# Autodesk Inventor assembly: Accelerator
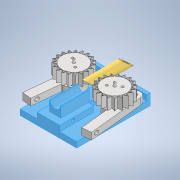
[picture p0: Inventor's stored thumbnail of the model, 180x180]
Saved by Autodesk Inventor 2021 (Build 250183000, 183)
## iProperties
Created: 2024-05-11
Part Number: Accelerator
Document SubType Name: Assembly
Designer: Lukas
Author: Lukas
## Documents named in this file (7)
- \\192.168.1.200\Storragepool\Datastorrage\CAD\Inventor 2019\Maccaroni-Gun\Inventor files\Accelerator.iam
- \\192.168.1.200\Storragepool\Datastorrage\CAD\Inventor 2019\Maccaroni-Gun\Inventor files\Motor_holder.ipt
- \\192.168.1.200\Storragepool\Datastorrage\CAD\Inventor 2019\Maccaroni-Gun\Inventor files\Motor_18mm.ipt
- \\192.168.1.200\Storragepool\Datastorrage\CAD\Inventor 2019\Maccaroni-Gun\Inventor files\Flywheel_base.ipt
- \\192.168.1.200\Storragepool\Datastorrage\CAD\Inventor 2019\Maccaroni-Gun\Inventor files\Antriebsrad.ipt
- \\192.168.1.200\Storragepool\Datastorrage\CAD\Inventor 2019\Maccaroni-Gun\Inventor files\Motor_holder_mirrored.ipt
- \\192.168.1.200\Storragepool\Datastorrage\CAD\Inventor 2019\Maccaroni-Gun\Inventor files\Maccaroni.ipt
## Components (8 placed, 6 different names)
1. Flywheel_base:1 — Mate:4, Mate:5, Mate:9, Mate:10, Mate:19, Angle:4, Angle:5, Flush:1, Flush:2, Flush:3
2. Motor_holder:1 — Mate:1, Mate:2, Mate:3, Mate:4, Mate:5, Rotation:1, Angle:4
3. Motor_holder_mirrored:1 — Mate:9, Mate:10, Mate:13, Mate:17, Mate:18, Rotation:1, Angle:5
4. Motor_18mm:1 — Mate:1, Mate:2, Mate:3, Mate:6, Mate:7, Mate:8
5. Motor_18mm:2 — Mate:13, Mate:14, Mate:15, Mate:16, Mate:17, Mate:18
6. Antriebsrad:1 — Mate:6, Mate:7, Mate:8
7. Antriebsrad:2 — Mate:14, Mate:15, Mate:16
8. Maccaroni:1 — Angle:3, Mate:19, Flush:4
## Relationships (25: Mate 17, Flush 4, Angle 3, RelateRotation 1)
- Mate:1: Motor_holder:1 ↔ Motor_18mm:1
- Mate:2: Motor_holder:1 ↔ Motor_18mm:1
- Mate:3: Motor_holder:1 ↔ Motor_18mm:1
- Mate:4: Flywheel_base:1 ↔ Motor_holder:1
- Mate:5: Flywheel_base:1 ↔ Motor_holder:1
- Mate:6: Motor_18mm:1 ↔ Antriebsrad:1
- Mate:7: Motor_18mm:1 ↔ Antriebsrad:1
- Mate:8: Motor_18mm:1 ↔ Antriebsrad:1
- Mate:9: Flywheel_base:1 ↔ Motor_holder_mirrored:1
- Mate:10: Flywheel_base:1 ↔ Motor_holder_mirrored:1
- Mate:13: Motor_holder_mirrored:1 ↔ Motor_18mm:2
- Mate:14: Motor_18mm:2 ↔ Antriebsrad:2
- Mate:15: Motor_18mm:2 ↔ Antriebsrad:2
- Mate:16: Motor_18mm:2 ↔ Antriebsrad:2
- Mate:17: Motor_holder_mirrored:1 ↔ Motor_18mm:2
- Mate:18: Motor_holder_mirrored:1 ↔ Motor_18mm:2
- Angle:3 (0 deg): Maccaroni:1
- Mate:19: Flywheel_base:1 ↔ Maccaroni:1
- Rotation:1 [RelateRotation] (1 ul): Motor_holder:1 ↔ Motor_holder_mirrored:1
- Angle:4 (0 deg): Flywheel_base:1 ↔ Motor_holder:1
- Angle:5 (0 deg): Flywheel_base:1 ↔ Motor_holder_mirrored:1
- Flush:1: Flywheel_base:1
- Flush:2: Flywheel_base:1
- Flush:3: Flywheel_base:1
- Flush:4 (-19 mm): Maccaroni:1
